# Autodesk Inventor assembly: POM_T5_03
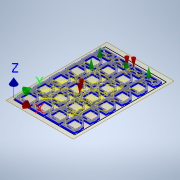
[picture p0: Inventor's stored thumbnail of the model, 180x180]
Saved by Autodesk Inventor 2022.3 (Build 263350000, 350)
## iProperties
Created: 2022-09-28
Part Number: POM_T5_03
Document SubType Name: Assembly
Designer: Masato
Author: Masato
## Documents named in this file (4)
- C:\Users\Masato\Documents\Inventor\Inventor for CIT Brains\SUSTAINA-OP - cam\Cam\POM_T5\OriginalMind_SR420\POM_T5_03.iam
- C:\Users\Masato\Documents\Inventor\Inventor for CIT Brains\SUSTAINA-OP - cam\Cam\DisposableBoard.ipt
- C:\Users\Masato\Documents\Inventor\Inventor for CIT Brains\SUSTAINA-OP - cam\UpperBody\Arm\ForeArm_diagonal.ipt
- C:\Users\Masato\Documents\Inventor\Inventor for CIT Brains\SUSTAINA-OP - cam\UpperBody\Head\Head_neck_diagonal.ipt
## Components (25 placed, 3 different names)
1. DisposableBoard:1 — フラッシュ:1, フラッシュ:2, フラッシュ:3, フラッシュ:4, Flush:5, Flush:6
2. ForeArm_diagonal:1 — Mate:1, Flush:5, Flush:6
3. ForeArm_diagonal:2
4. ForeArm_diagonal:3
5. ForeArm_diagonal:4
6. ForeArm_diagonal:5
7. ForeArm_diagonal:6
8. ForeArm_diagonal:7
9. ForeArm_diagonal:8
10. ForeArm_diagonal:9
11. ForeArm_diagonal:10
12. ForeArm_diagonal:11
13. ForeArm_diagonal:12
14. ForeArm_diagonal:13
15. ForeArm_diagonal:14
16. ForeArm_diagonal:15
17. ForeArm_diagonal:16
18. ForeArm_diagonal:17 — Flush:7, Mate:3
19. ForeArm_diagonal:18
20. ForeArm_diagonal:19
21. ForeArm_diagonal:20
22. Head_neck_diagonal:1 — Mate:2, Flush:7, Mate:3
23. Head_neck_diagonal:2
24. Head_neck_diagonal:3
25. Head_neck_diagonal:4
## Component patterns: (20 elements, first: ForeArm_diagonal:1), (4 elements, first: Head_neck_diagonal:1)
## Relationships (10: Flush 7, Mate 3)
- フラッシュ:1 [Flush]: DisposableBoard:1
- フラッシュ:2 [Flush]: DisposableBoard:1
- フラッシュ:3 [Flush]: DisposableBoard:1
- フラッシュ:4 [Flush]: DisposableBoard:1
- Mate:1: ForeArm_diagonal:1
- Flush:5 (-2 mm): DisposableBoard:1 ↔ ForeArm_diagonal:1
- Flush:6 (2 mm): DisposableBoard:1 ↔ ForeArm_diagonal:1
- Mate:2: Head_neck_diagonal:1
- Flush:7: ForeArm_diagonal:17 ↔ Head_neck_diagonal:1
- Mate:3 (2.1 mm): ForeArm_diagonal:17 ↔ Head_neck_diagonal:1
